# Autodesk Inventor assembly: PitchMotor
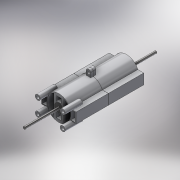
[picture p0: Inventor's stored thumbnail of the model, 180x180]
Saved by Autodesk Inventor 2018 (Build 220112000, 112)
## iProperties
Created: 2018-03-13
Part Number: PitchMotor
Document SubType Name: Assembly
Designer: mansu
Sending System: SolidWorks 2017
Last Author: leoli
Last Saved: 2018-03-15
Author: mansu
## Documents named in this file (7)
- F:\OneDrive\Documents\2018 UBC\ELEC 391\Controller\cad\release\PitchMotor.iam
- F:\OneDrive\Documents\2018 UBC\ELEC 391\Motor\SolidWorks\Pitch\pitch_StatorShell_v3.ipt
- F:\OneDrive\Documents\2018 UBC\ELEC 391\Motor\SolidWorks\Pitch\pitch_StatorShell_v2_attachment.ipt
- F:\OneDrive\Documents\2018 UBC\ELEC 391\Motor\SolidWorks\Pitch\pitch_bearings.ipt
- F:\OneDrive\Documents\2018 UBC\ELEC 391\Motor\SolidWorks\Pitch\pitch_shaft.ipt
- F:\OneDrive\Documents\2018 UBC\ELEC 391\Motor\SolidWorks\Pitch\pitch_RotorCore.ipt
- F:\OneDrive\Documents\2018 UBC\ELEC 391\Motor\SolidWorks\Pitch\pitch_commutator_attachment1.ipt
## Components (7 placed, 6 different names)
1. pitch_StatorShell_v3:1 — Mate:2, Flush:2, Mate:7, Mate:8, Mate:9
2. pitch_StatorShell_v2_attachment:2 — Mate:3, Flush:1, Mate:8, Mate:9
3. pitch_bearings:1 — Mate:3, Flush:1, Mate:5, Flush:3
4. pitch_bearings:2 — Mate:2, Flush:2, Mate:4
5. pitch_shaft:1 — Mate:1, Mate:4, Mate:5, Mate:6, Flush:3
6. pitch_RotorCore:1 — Mate:1, Mate:7
7. pitch_commutator_attachment1:1 — Mate:6
## Relationships (12: Mate 9, Flush 3)
- Mate:1: pitch_shaft:1 ↔ pitch_RotorCore:1
- Mate:2: pitch_StatorShell_v3:1 ↔ pitch_bearings:2
- Mate:3: pitch_StatorShell_v2_attachment:2 ↔ pitch_bearings:1
- Flush:1: pitch_StatorShell_v2_attachment:2 ↔ pitch_bearings:1
- Flush:2: pitch_StatorShell_v3:1 ↔ pitch_bearings:2
- Mate:4: pitch_bearings:2 ↔ pitch_shaft:1
- Mate:5: pitch_bearings:1 ↔ pitch_shaft:1
- Mate:6: pitch_shaft:1 ↔ pitch_commutator_attachment1:1
- Mate:7 (1 mm): pitch_StatorShell_v3:1 ↔ pitch_RotorCore:1
- Mate:8: pitch_StatorShell_v3:1 ↔ pitch_StatorShell_v2_attachment:2
- Mate:9 (0.1 mm): pitch_StatorShell_v3:1 ↔ pitch_StatorShell_v2_attachment:2
- Flush:3 (40 mm): pitch_bearings:1 ↔ pitch_shaft:1
